# Autodesk Inventor assembly: Asem
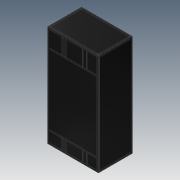
[picture p0: Inventor's stored thumbnail of the model, 180x180]
Saved by Autodesk Inventor 2020 (Build 240168000, 168)
## iProperties
Created: 2021-02-24
Part Number: Asem
Document SubType Name: Assembly
Designer: magnarecta
Author: magnarecta
## Documents named in this file (15)
- C:\Users\lvglv\Documents\GitHub\Eto_Project\Hardware\Asem\Asem.iam
- C:\Users\lvglv\Documents\GitHub\Eto_Project\Hardware\Parts\MISUMI\HFS6-3030-1500_Autodesk_Inventor_2020_20210225\HFS6-3030-1500.ipt
- C:\Users\lvglv\Documents\GitHub\Eto_Project\Hardware\Parts\MISUMI\HFS6-3030-690_Autodesk_Inventor_2020_20210225\HFS6-3030-690.ipt
- C:\Users\lvglv\Documents\GitHub\Eto_Project\Hardware\Parts\MISUMI\HFS6-3030-440_Autodesk_Inventor_2020_20210225\HFS6-3030-440.ipt
- C:\Users\lvglv\Documents\GitHub\Eto_Project\Hardware\Asem\CCM_Unit.iam
- C:\Users\lvglv\Documents\GitHub\Eto_Project\Hardware\Parts\MISUMI\HFS6-3030-223_Autodesk_Inventor_2020_20210225\HFS6-3030-223.ipt
- C:\Users\lvglv\Documents\GitHub\Eto_Project\Hardware\Parts\MISUMI\HFS6-3030-140_Autodesk_Inventor_2020_20210225\HFS6-3030-140.ipt
- C:\Users\lvglv\Documents\GitHub\Eto_Project\Hardware\Parts\Meviy\Dragchain_Guide.ipt
- C:\Users\lvglv\Documents\GitHub\Eto_Project\Hardware\Parts\MISUMI\HFS6-3030-1440_Autodesk_Inventor_2020_20210225\HFS6-3030-1440.ipt
- C:\Users\lvglv\Documents\GitHub\Eto_Project\Hardware\Parts\Meviy\Plate\Panel_A.ipt
- C:\Users\lvglv\Documents\GitHub\Eto_Project\Hardware\Parts\Meviy\Plate\Panel_B.ipt
- C:\Users\lvglv\Documents\GitHub\Eto_Project\Hardware\Parts\Meviy\Plate\Panel_C.ipt
- C:\Users\lvglv\Documents\GitHub\Eto_Project\Hardware\Parts\Meviy\Plate\Panel_D.ipt
- C:\Users\lvglv\Documents\GitHub\Eto_Project\Hardware\Parts\Meviy\Plate\Panel_E.ipt
- C:\Users\lvglv\Documents\GitHub\Eto_Project\Hardware\Parts\Grabcad\elecrow-10-1-screen-monitor-1.snapshot.2\elecrow 10.1 inch.ipt
## Components (36 placed, 14 different names)
1. HFS6-3030-1500:1 — フラッシュ:1, フラッシュ:2, フラッシュ:5, メイト:1, フラッシュ:6, フラッシュ:7, メイト:2, フラッシュ:9, フラッシュ:10, フラッシュ:18, フラッシュ:21, フラッシュ:25, メイト:20, フラッシュ:58, メイト:37, メイト:38
2. HFS6-3030-1500:2 — フラッシュ:2, フラッシュ:5, メイト:1, フラッシュ:8, メイト:3, メイト:4, フラッシュ:11, フラッシュ:12, フラッシュ:20, メイト:10, フラッシュ:24, メイト:12, メイト:13, フラッシュ:26
3. HFS6-3030-1500:3 — フラッシュ:3, フラッシュ:4, フラッシュ:8, メイト:5, フラッシュ:13, フラッシュ:14, メイト:6, フラッシュ:15, フラッシュ:16, メイト:34
4. HFS6-3030-1500:4 — フラッシュ:1, フラッシュ:3, フラッシュ:4, フラッシュ:6, フラッシュ:7, メイト:2, フラッシュ:55, メイト:41
5. HFS6-3030-690:1 — メイト:3, フラッシュ:9, フラッシュ:10, メイト:7, フラッシュ:17, メイト:8, フラッシュ:19, メイト:15, メイト:18, フラッシュ:33, メイト:19
6. HFS6-3030-690:2 — メイト:4, フラッシュ:11, フラッシュ:12, メイト:9, フラッシュ:22, フラッシュ:23, メイト:11, 角度:1, メイト:14, フラッシュ:28, メイト:29, フラッシュ:57
7. HFS6-3030-690:3 — メイト:5, フラッシュ:13, フラッシュ:14, メイト:28, メイト:30
8. HFS6-3030-690:4 — メイト:6, フラッシュ:15, フラッシュ:16, メイト:31
9. HFS6-3030-440:1 — メイト:7, フラッシュ:17, フラッシュ:20
10. HFS6-3030-440:2 — メイト:8, フラッシュ:18, フラッシュ:19, フラッシュ:59
11. HFS6-3030-440:3 — メイト:9, フラッシュ:21, フラッシュ:22, メイト:27, フラッシュ:54, フラッシュ:56
12. HFS6-3030-440:4 — メイト:10, フラッシュ:23, フラッシュ:24
13. CCM_Unit:1 [sub-assembly] — メイト:11, 角度:1, フラッシュ:27, フラッシュ:34, フラッシュ:36, メイト:24, メイト:25, メイト:26, メイト:45, メイト:46, メイト:47
14. HFS6-3030-690:5 — メイト:12, フラッシュ:25, メイト:14, フラッシュ:43, メイト:21
15. HFS6-3030-690:6 — メイト:13, フラッシュ:26, メイト:15, フラッシュ:35
16. HFS6-3030-223:1 — フラッシュ:31, フラッシュ:32, メイト:17, メイト:18, フラッシュ:47
17. HFS6-3030-223:2 — フラッシュ:31, フラッシュ:32, メイト:17, フラッシュ:33, フラッシュ:34, メイト:20, フラッシュ:44
18. HFS6-3030-223:3 — フラッシュ:29, フラッシュ:30, メイト:16, フラッシュ:46
19. HFS6-3030-223:4 — フラッシュ:29, フラッシュ:30, メイト:16, メイト:19, フラッシュ:35, フラッシュ:36, フラッシュ:45
20. HFS6-3030-140:1 — フラッシュ:37, フラッシュ:42, メイト:21, フラッシュ:44
21. HFS6-3030-140:2 — フラッシュ:37, フラッシュ:38, フラッシュ:41, フラッシュ:42, フラッシュ:43, フラッシュ:46
22. HFS6-3030-140:3 — フラッシュ:38, フラッシュ:39, フラッシュ:40, フラッシュ:41, フラッシュ:47
23. HFS6-3030-140:4 — フラッシュ:39, フラッシュ:40, フラッシュ:45
24. Dragchain_Guide:1 — メイト:23, フラッシュ:50, メイト:24, フラッシュ:51
25. Dragchain_Guide:3 — メイト:23, フラッシュ:50, フラッシュ:51, メイト:25, メイト:26
26. HFS6-3030-1440:1 — フラッシュ:52, フラッシュ:53, メイト:37
27. HFS6-3030-1440:2 — フラッシュ:52, フラッシュ:53, メイト:27, フラッシュ:54, フラッシュ:61
28. Panel_A:1 — メイト:28, フラッシュ:55, フラッシュ:56, メイト:32, メイト:36, メイト:43
29. Panel_A:2 — メイト:29, フラッシュ:57, フラッシュ:58, メイト:33, メイト:39
30. Panel_B:1 — メイト:30, フラッシュ:60, メイト:33, メイト:40, メイト:42
31. Panel_B:2 — メイト:31, メイト:32, フラッシュ:59, フラッシュ:60, メイト:35
32. Panel_C:1 — メイト:34, メイト:35, メイト:36
33. Panel_D:1 — メイト:38, メイト:39, メイト:40
34. Panel_E:1 — メイト:41, メイト:42, メイト:43, フラッシュ:61
35. elecrow 10.1 inch:1 — フラッシュ:62, 角度:2, フラッシュ:63, メイト:44, メイト:45, メイト:46
36. elecrow 10.1 inch:2 — フラッシュ:62, 角度:2, フラッシュ:63, メイト:44, メイト:47
## Relationships (109: Flush 61, Mate 46, Angle 2)
- フラッシュ:1 [Flush]: HFS6-3030-1500:1 ↔ HFS6-3030-1500:4
- フラッシュ:2 [Flush]: HFS6-3030-1500:1 ↔ HFS6-3030-1500:2
- フラッシュ:3 [Flush]: HFS6-3030-1500:3 ↔ HFS6-3030-1500:4
- フラッシュ:4 [Flush]: HFS6-3030-1500:3 ↔ HFS6-3030-1500:4
- フラッシュ:5 [Flush]: HFS6-3030-1500:1 ↔ HFS6-3030-1500:2
- メイト:1 [Mate] (-750 mm): HFS6-3030-1500:1 ↔ HFS6-3030-1500:2
- フラッシュ:6 [Flush]: HFS6-3030-1500:1 ↔ HFS6-3030-1500:4
- フラッシュ:7 [Flush]: HFS6-3030-1500:1 ↔ HFS6-3030-1500:4
- フラッシュ:8 [Flush]: HFS6-3030-1500:2 ↔ HFS6-3030-1500:3
- メイト:2 [Mate] (-500 mm): HFS6-3030-1500:1 ↔ HFS6-3030-1500:4
- メイト:3 [Mate]: HFS6-3030-1500:2 ↔ HFS6-3030-690:1
- フラッシュ:9 [Flush]: HFS6-3030-1500:1 ↔ HFS6-3030-690:1
- フラッシュ:10 [Flush]: HFS6-3030-1500:1 ↔ HFS6-3030-690:1
- メイト:4 [Mate]: HFS6-3030-1500:2 ↔ HFS6-3030-690:2
- フラッシュ:11 [Flush]: HFS6-3030-1500:2 ↔ HFS6-3030-690:2
- フラッシュ:12 [Flush]: HFS6-3030-1500:2 ↔ HFS6-3030-690:2
- メイト:5 [Mate]: HFS6-3030-1500:3 ↔ HFS6-3030-690:3
- フラッシュ:13 [Flush]: HFS6-3030-1500:3 ↔ HFS6-3030-690:3
- フラッシュ:14 [Flush]: HFS6-3030-1500:3 ↔ HFS6-3030-690:3
- メイト:6 [Mate]: HFS6-3030-1500:3 ↔ HFS6-3030-690:4
- フラッシュ:15 [Flush]: HFS6-3030-1500:3 ↔ HFS6-3030-690:4
- フラッシュ:16 [Flush]: HFS6-3030-1500:3 ↔ HFS6-3030-690:4
- メイト:7 [Mate]: HFS6-3030-690:1 ↔ HFS6-3030-440:1
- フラッシュ:17 [Flush]: HFS6-3030-690:1 ↔ HFS6-3030-440:1
- メイト:8 [Mate]: HFS6-3030-690:1 ↔ HFS6-3030-440:2
- フラッシュ:18 [Flush]: HFS6-3030-1500:1 ↔ HFS6-3030-440:2
- フラッシュ:19 [Flush]: HFS6-3030-690:1 ↔ HFS6-3030-440:2
- フラッシュ:20 [Flush]: HFS6-3030-1500:2 ↔ HFS6-3030-440:1
- メイト:9 [Mate]: HFS6-3030-690:2 ↔ HFS6-3030-440:3
- フラッシュ:21 [Flush]: HFS6-3030-1500:1 ↔ HFS6-3030-440:3
- フラッシュ:22 [Flush]: HFS6-3030-690:2 ↔ HFS6-3030-440:3
- メイト:10 [Mate]: HFS6-3030-1500:2 ↔ HFS6-3030-440:4
- フラッシュ:23 [Flush]: HFS6-3030-690:2 ↔ HFS6-3030-440:4
- フラッシュ:24 [Flush]: HFS6-3030-1500:2 ↔ HFS6-3030-440:4
- メイト:11 [Mate] (2 mm): HFS6-3030-690:2 ↔ CCM_Unit:1
- 角度:1 [Angle] (0 deg): HFS6-3030-690:2 ↔ CCM_Unit:1
- メイト:12 [Mate]: HFS6-3030-1500:2 ↔ HFS6-3030-690:5
- フラッシュ:25 [Flush]: HFS6-3030-1500:1 ↔ HFS6-3030-690:5
- メイト:13 [Mate]: HFS6-3030-1500:2 ↔ HFS6-3030-690:6
- フラッシュ:26 [Flush]: HFS6-3030-1500:2 ↔ HFS6-3030-690:6
- メイト:14 [Mate] (-200 mm): HFS6-3030-690:2 ↔ HFS6-3030-690:5
- メイト:15 [Mate] (-283 mm): HFS6-3030-690:1 ↔ HFS6-3030-690:6
- フラッシュ:27 [Flush] (-10 mm): CCM_Unit:1
- フラッシュ:28 [Flush] (70 mm): HFS6-3030-690:2
- フラッシュ:29 [Flush]: HFS6-3030-223:3 ↔ HFS6-3030-223:4
- フラッシュ:30 [Flush]: HFS6-3030-223:3 ↔ HFS6-3030-223:4
- メイト:16 [Mate] (20 mm): HFS6-3030-223:3 ↔ HFS6-3030-223:4
- フラッシュ:31 [Flush]: HFS6-3030-223:1 ↔ HFS6-3030-223:2
- フラッシュ:32 [Flush]: HFS6-3030-223:1 ↔ HFS6-3030-223:2
- メイト:17 [Mate] (20 mm): HFS6-3030-223:1 ↔ HFS6-3030-223:2
- メイト:18 [Mate]: HFS6-3030-690:1 ↔ HFS6-3030-223:1
- フラッシュ:33 [Flush]: HFS6-3030-690:1 ↔ HFS6-3030-223:2
- フラッシュ:34 [Flush] (-7.5 mm): CCM_Unit:1 ↔ HFS6-3030-223:2
- メイト:19 [Mate]: HFS6-3030-690:1 ↔ HFS6-3030-223:4
- フラッシュ:35 [Flush]: HFS6-3030-690:6 ↔ HFS6-3030-223:4
- フラッシュ:36 [Flush]: CCM_Unit:1 ↔ HFS6-3030-223:4
- メイト:20 [Mate] (170 mm): HFS6-3030-1500:1 ↔ HFS6-3030-223:2
- フラッシュ:37 [Flush]: HFS6-3030-140:1 ↔ HFS6-3030-140:2
- フラッシュ:38 [Flush]: HFS6-3030-140:2 ↔ HFS6-3030-140:3
- フラッシュ:39 [Flush]: HFS6-3030-140:3 ↔ HFS6-3030-140:4
- フラッシュ:40 [Flush]: HFS6-3030-140:3 ↔ HFS6-3030-140:4
- フラッシュ:41 [Flush]: HFS6-3030-140:2 ↔ HFS6-3030-140:3
- フラッシュ:42 [Flush]: HFS6-3030-140:1 ↔ HFS6-3030-140:2
- フラッシュ:43 [Flush]: HFS6-3030-690:5 ↔ HFS6-3030-140:2
- メイト:21 [Mate]: HFS6-3030-690:5 ↔ HFS6-3030-140:1
- フラッシュ:44 [Flush]: HFS6-3030-223:2 ↔ HFS6-3030-140:1
- フラッシュ:45 [Flush]: HFS6-3030-223:4 ↔ HFS6-3030-140:4
- フラッシュ:46 [Flush]: HFS6-3030-223:3 ↔ HFS6-3030-140:2
- フラッシュ:47 [Flush]: HFS6-3030-223:1 ↔ HFS6-3030-140:3
- メイト:23 [Mate]: Dragchain_Guide:1 ↔ Dragchain_Guide:3
- フラッシュ:50 [Flush]: Dragchain_Guide:1 ↔ Dragchain_Guide:3
- メイト:24 [Mate]: CCM_Unit:1 ↔ Dragchain_Guide:1
- フラッシュ:51 [Flush]: Dragchain_Guide:1 ↔ Dragchain_Guide:3
- メイト:25 [Mate]: CCM_Unit:1 ↔ Dragchain_Guide:3
- メイト:26 [Mate] (-13 mm): CCM_Unit:1 ↔ Dragchain_Guide:3
- フラッシュ:52 [Flush]: HFS6-3030-1440:1 ↔ HFS6-3030-1440:2
- フラッシュ:53 [Flush]: HFS6-3030-1440:1 ↔ HFS6-3030-1440:2
- メイト:27 [Mate]: HFS6-3030-440:3 ↔ HFS6-3030-1440:2
- フラッシュ:54 [Flush]: HFS6-3030-440:3 ↔ HFS6-3030-1440:2
- メイト:28 [Mate]: HFS6-3030-690:3 ↔ Panel_A:1
- フラッシュ:55 [Flush]: HFS6-3030-1500:4 ↔ Panel_A:1
- フラッシュ:56 [Flush]: HFS6-3030-440:3 ↔ Panel_A:1
- メイト:29 [Mate]: HFS6-3030-690:2 ↔ Panel_A:2
- フラッシュ:57 [Flush]: HFS6-3030-690:2 ↔ Panel_A:2
- フラッシュ:58 [Flush]: HFS6-3030-1500:1 ↔ Panel_A:2
- メイト:30 [Mate]: HFS6-3030-690:3 ↔ Panel_B:1
- メイト:31 [Mate]: HFS6-3030-690:4 ↔ Panel_B:2
- メイト:32 [Mate]: Panel_A:1 ↔ Panel_B:2
- フラッシュ:59 [Flush]: HFS6-3030-440:2 ↔ Panel_B:2
- フラッシュ:60 [Flush]: Panel_B:1 ↔ Panel_B:2
- メイト:33 [Mate]: Panel_A:2 ↔ Panel_B:1
- メイト:34 [Mate]: HFS6-3030-1500:3 ↔ Panel_C:1
- メイト:35 [Mate]: Panel_B:2 ↔ Panel_C:1
- メイト:36 [Mate]: Panel_A:1 ↔ Panel_C:1
- メイト:37 [Mate] (150 mm): HFS6-3030-1500:1 ↔ HFS6-3030-1440:1
- メイト:38 [Mate]: HFS6-3030-1500:1 ↔ Panel_D:1
- メイト:39 [Mate]: Panel_A:2 ↔ Panel_D:1
- メイト:40 [Mate]: Panel_B:1 ↔ Panel_D:1
- メイト:41 [Mate]: HFS6-3030-1500:4 ↔ Panel_E:1
- メイト:42 [Mate]: Panel_B:1 ↔ Panel_E:1
- メイト:43 [Mate]: Panel_A:1 ↔ Panel_E:1
- フラッシュ:61 [Flush]: HFS6-3030-1440:2 ↔ Panel_E:1
- フラッシュ:62 [Flush]: elecrow 10.1 inch:1 ↔ elecrow 10.1 inch:2
- 角度:2 [Angle] (0 deg): elecrow 10.1 inch:1 ↔ elecrow 10.1 inch:2
- フラッシュ:63 [Flush]: elecrow 10.1 inch:1 ↔ elecrow 10.1 inch:2
- メイト:44 [Mate] (2 mm): elecrow 10.1 inch:1 ↔ elecrow 10.1 inch:2
- メイト:45 [Mate] (-15 mm): CCM_Unit:1 ↔ elecrow 10.1 inch:1
- メイト:46 [Mate] (2 mm): CCM_Unit:1 ↔ elecrow 10.1 inch:1
- メイト:47 [Mate] (30 mm): CCM_Unit:1 ↔ elecrow 10.1 inch:2
